# Autodesk Inventor assembly: !conveyer_box
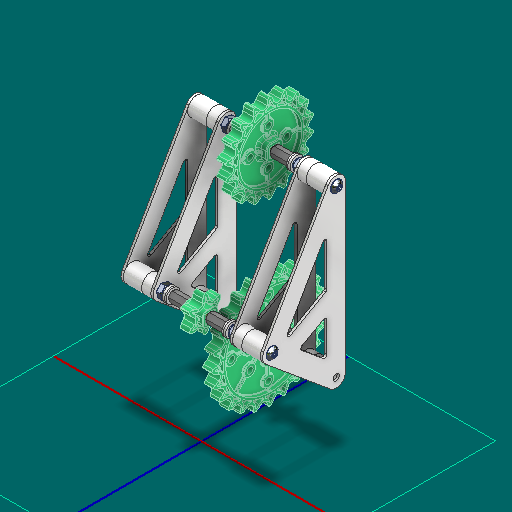
[picture p0: Inventor's stored thumbnail of the model, 512x512]
Saved by Autodesk Inventor 2025 (Build 290162000, 162)
## iProperties
Created: 2024-08-19
Part Number: !conveyer_box
Document SubType Name: Assembly
Designer: averey
Author: averey
## Documents named in this file (10)
- C:\Users\avere\vex_robotics_high_stakes\hardware\cad\ATLAS\tower\conveyer_box\!conveyer_box.iam
- C:\Users\avere\vex_robotics_high_stakes\hardware\cad\ATLAS\tower\conveyer_box\structure.iam
- structure.iam
- C:\Users\avere\vex_robotics_high_stakes\hardware\cad\ATLAS\tower\conveyer_box\structure_mirrored\structure_mirrored.iam
- C:\Users\avere\vex_robotics_high_stakes\hardware\cad\VEX-CAD-Inventor\Motion\Sprockets\9P Sprocket.iam
- C:\Users\avere\vex_robotics_high_stakes\hardware\cad\VEX-CAD-Inventor\Motion\Sprockets\9P Sprocket\9P 18T Sprocket, No Insert.iam
- C:\Users\avere\vex_robotics_high_stakes\hardware\cad\VEX-CAD-Inventor\Motion\Sprockets\9P Sprocket\9P 24T Sprocket, No Insert.iam
- C:\Users\avere\vex_robotics_high_stakes\hardware\cad\VEX-CAD-Inventor\Motion\Sprockets\9P Sprocket\9P 6T Sprocket, No Insert.iam
- C:\Users\avere\vex_robotics_high_stakes\hardware\cad\VEX-CAD-Inventor\Motion\Sprockets\6P Sprocket\6P 8T Sprocket, No Insert.iam
- C:\Users\avere\vex_robotics_high_stakes\hardware\cad\VEX-CAD-Inventor\Motion\Sprockets\6P Sprocket.iam
## Components (7 placed, 6 different names)
1. structure:1 [sub-assembly] — Insert:1, Mate:1, Mate:2, Mate:3, Insert:3, Mate:4, Insert:4
2. structure_mirrored:1 [sub-assembly] — Insert:1, Mate:1, Angle:1
3. 9P 18T Sprocket, No Insert:3 [sub-assembly] — Insert:3
4. 9P 24T Sprocket, No Insert:4 [sub-assembly] — Mate:4, Flush:1, Insert:5, Insert:6
5. 9P 6T Sprocket, No Insert:5 [sub-assembly] — Insert:4, Flush:1
6. 6P 8T Sprocket, No Insert:1 [sub-assembly] — Insert:5
7. 6P 8T Sprocket, No Insert:2 [sub-assembly] — Insert:6
## Relationships (11: Insert 5, Mate 4, Angle 1, Flush 1)
- Insert:1 (53.2035 mm): structure:1 ↔ structure_mirrored:1
- Mate:1: structure:1 ↔ structure_mirrored:1
- Mate:2: structure:1
- Mate:3 (26.6017 mm): structure:1
- Angle:1 (0 deg): structure_mirrored:1
- Insert:3: structure:1 ↔ 9P 18T Sprocket, No Insert:3
- Mate:4: structure:1 ↔ 9P 24T Sprocket, No Insert:4
- Insert:4: structure:1 ↔ 9P 6T Sprocket, No Insert:5
- Flush:1: 9P 24T Sprocket, No Insert:4 ↔ 9P 6T Sprocket, No Insert:5
- Insert:5: 9P 24T Sprocket, No Insert:4 ↔ 6P 8T Sprocket, No Insert:1
- Insert:6: 9P 24T Sprocket, No Insert:4 ↔ 6P 8T Sprocket, No Insert:2
